# Autodesk Inventor assembly: Robot
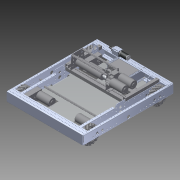
[picture p0: Inventor's stored thumbnail of the model, 180x180]
Saved by Autodesk Inventor 2015 SP1 (Build 190203100, 203)
## iProperties
Created: 2015-01-10
Part Number: Robot
Document SubType Name: Assembly
Designer: Jarod
Author: Jarod
## Documents named in this file (29)
- C:\Users\Jarod\Documents\Westview\Robotics\FRC\2015\CAD\Robot\Chassis\Chassis.iam
- C:\Users\Jarod\Documents\Westview\Robotics\FRC\2015\CAD\Robot\Chassis\Imported Components\AM14U2 End Sheet\AM14U2 End Sheet.ipt
- C:\Users\Jarod\Documents\Westview\Robotics\FRC\2015\CAD\Robot\Chassis\Imported Components\AM14U2 Inside Sheet\AM14U2 Inside Sheet.ipt
- C:\Users\Jarod\Documents\Westview\Robotics\FRC\2015\CAD\Robot\Chassis\Imported Components\AM14U2 Outside Sheet\AM14U2 Outside Sheet.ipt
- C:\Users\Jarod\Documents\Westview\Robotics\FRC\2015\CAD\Robot\Chassis\Imported Components\hub hex 0.5in\hub hex 0.5in.ipt
- C:\Users\Jarod\Documents\Westview\Robotics\FRC\2015\CAD\Robot\Chassis\Imported Components\Toughbox nano hex\Toughbox nano hex.iam
- C:\Users\Jarod\Documents\Westview\Robotics\FRC\2015\CAD\Robot\Chassis\ToughBox Nano Mounting Plate.ipt
- C:\Users\Jarod\Documents\Westview\Robotics\FRC\2015\CAD\Robot\Chassis\Imported Components\mecanum 6in left\mecanum 6in left.iam
- C:\Users\Jarod\Documents\Westview\Robotics\FRC\2015\CAD\Robot\Chassis\Imported Components\mecanum 6in right\mecanum 6in right.iam
- C:\Users\Jarod\Documents\Westview\Robotics\FRC\2015\CAD\Robot\Chassis\Imported Components\Battery Holder\Battery Holder.iam
- C:\Users\Jarod\Documents\Westview\Robotics\FRC\2015\CAD\Robot\Chassis\battery.ipt
- C:\Users\Jarod\Documents\Westview\Robotics\FRC\2015\CAD\Robot\Chassis\polycarb base.ipt
- C:\Users\Jarod\Documents\Westview\Robotics\FRC\2015\CAD\Robot\Chassis\churro.ipt
- C:\Users\Jarod\Documents\Westview\Robotics\FRC\2015\CAD\Robot\Chassis\churro long.ipt
- C:\Users\Jarod\Documents\Westview\Robotics\FRC\2015\CAD\Robot\Chassis\Imported Components\Versaplanetary Gearbox\Versaplanetary Gearbox.iam
- C:\Users\Jarod\Documents\Westview\Robotics\FRC\2015\CAD\Robot\Chassis\Imported Components\0.5 Hex #25 Chain 16t Sprocket\0.5 Hex #25 Chain 16t Sprocket.ipt
- C:\Users\Jarod\Documents\Westview\Robotics\FRC\2015\CAD\Robot\Chassis\Imported Components\0.5 Hex Shaft Collar\0.5 Hex Shaft Collar.ipt
- C:\Users\Jarod\Documents\Westview\Robotics\FRC\2015\CAD\Robot\Chassis\mounting block.ipt
- C:\Users\Jarod\Documents\Westview\Robotics\FRC\2015\CAD\Robot\Chassis\Imported Components\Bearing Side Gusset\Bearing Side Gusset.ipt
- C:\Users\Jarod\Documents\Westview\Robotics\FRC\2015\CAD\Robot\Chassis\mounting block long.ipt
- C:\Users\Jarod\Documents\Westview\Robotics\FRC\2015\CAD\Robot\Chassis\Imported Components\Toughbox-mini\Toughbox-mini.iam
- C:\Users\Jarod\Documents\Westview\Robotics\FRC\2015\CAD\Robot\Chassis\Imported Components\Toughbox-mini\Toughbox-mini_d02.ipt
- C:\Users\Jarod\Documents\Westview\Robotics\FRC\2015\CAD\Robot\Chassis\Imported Components\0.5 Hex Bearing\0.5 Hex Bearing.ipt
- C:\Users\Jarod\Documents\Westview\Robotics\FRC\2015\CAD\Robot\Chassis\Imported Components\0.5 hex coupler\0.5 hex coupler.iam
- C:\Users\Jarod\Documents\Westview\Robotics\FRC\2015\CAD\Robot\Chassis\Imported Components\Toughbox nano hex\CIM motor.ipt
- C:\Users\Jarod\Documents\Westview\Robotics\FRC\2015\CAD\Robot\Chassis\churro gearbox support.ipt
- C:\Users\Jarod\Documents\Westview\Robotics\FRC\2015\CAD\Robot\Chassis\0.5 hex shaft.ipt
- C:\Users\Jarod\Documents\Westview\Robotics\FRC\2015\CAD\Robot\Chassis\2in spool roller.ipt
- C:\Users\Jarod\Documents\Westview\Robotics\FRC\2015\CAD\Robot\Chassis\spool roller hub.ipt
## Components (53 placed, 28 different names)
1. AM14U2 End Sheet:1 — Mate:1, Flush:1, Flush:2, Mate:2, Mate:12, Mate:13, Mate:14, Mate:15, Mate:16, Mate:17, Mate:18, Mate:54, Mate:56, Mate:58, Mate:59, Mate:60, Mate:61, Mate:72, Mate:73
2. AM14U2 End Sheet:2 — Mate:19, Mate:20, Mate:21, Mate:55, Mate:57, Mate:66, Mate:67, Mate:68, Mate:70, Mate:94
3. AM14U2 Inside Sheet:1 — Mate:12, Mate:47, Mate:49, Flush:7, Flush:8, Mate:60, Mate:61, Mate:62, Mate:63, Flush:11, Mate:74, Mate:75, Mate:78, Mate:79, Mate:82, Mate:83, Mate:84, Mate:85, Mate:122, Mate:139, Mate:151, Mate:152, Mate:153, Mate:155, Mate:156
4. AM14U2 Inside Sheet:2 — Mate:2, Mate:46, Mate:48, Flush:9, Flush:10, Mate:58, Mate:59, Mate:64, Mate:65, Mate:76, Mate:77, Mate:80, Mate:81, Mate:125, Mate:140, Mate:154, Mate:157, Mate:158
5. AM14U2 Outside Sheet:1 — Mate:13, Mate:14, Mate:15, Mate:19, Mate:20, Mate:21
6. AM14U2 Outside Sheet:2 — Mate:16, Mate:17, Mate:18
7. churro:1 — Mate:74, Mate:79
8. churro:2 — Mate:75, Mate:78
9. churro:3 — Mate:76, Mate:81
10. churro:4 — Mate:77, Mate:80
11. churro long:1 — Mate:82, Mate:84
12. churro long:2 — Mate:83, Mate:85
13. Toughbox nano hex:1 [sub-assembly] — Mate:23, Mate:25, Mate:38, Flush:3, Mate:39, Mate:54, Flush:7
14. Toughbox nano hex:2 [sub-assembly] — Mate:26, Mate:29, Mate:40, Flush:4, Mate:41, Mate:55, Flush:8
15. Toughbox nano hex:3 [sub-assembly] — Mate:30, Mate:33, Mate:44, Flush:6, Mate:45, Flush:9, Mate:56
16. Toughbox nano hex:4 [sub-assembly] — Mate:36, Mate:42, Flush:5, Mate:43, Mate:57, Flush:10
17. ToughBox Nano Mounting Plate:1 — Mate:38, Flush:3, Mate:39, Mate:47
18. ToughBox Nano Mounting Plate:2 — Mate:40, Flush:4, Mate:41, Mate:49
19. ToughBox Nano Mounting Plate:3 — Mate:44, Flush:6, Mate:45, Mate:46
20. ToughBox Nano Mounting Plate:4 — Mate:42, Flush:5, Mate:43, Mate:48
21. hub hex 0.5in:1 — Mate:23, Mate:24, Mate:63
22. hub hex 0.5in:2 — Mate:26, Mate:28, Mate:62
23. hub hex 0.5in:3 — Mate:30, Mate:32, Mate:64
24. hub hex 0.5in:4 — Mate:34, Mate:35, Mate:36, Mate:65
25. mecanum 6in left:1 [sub-assembly] — Mate:24, Mate:25
26. mecanum 6in left:2 [sub-assembly] — Mate:34, Mate:35
27. mecanum 6in right:1 [sub-assembly] — Mate:28, Mate:29
28. mecanum 6in right:2 [sub-assembly] — Mate:32, Mate:33
29. Battery Holder:1 [sub-assembly] — Mate:66, Mate:67, Mate:68, Mate:69, Mate:71, Mate:114, Mate:115
30. battery:1 — Mate:69, Mate:70, Mate:71
31. polycarb base:1 — Mate:72, Flush:11, Mate:73
32. Versaplanetary Gearbox:1 [sub-assembly] — Mate:94, Mate:97, Mate:100, Mate:114, Mate:115
33. 0.5 Hex #25 Chain 16t Sprocket:1 — Mate:97, Mate:98, Mate:99, Mate:100
34. 0.5 Hex Shaft Collar:1 — Mate:98, Mate:99
35. mounting block:1 — Mate:122, Mate:131, Mate:132, Mate:133, Mate:155, Mate:156
36. mounting block:2 — Mate:125, Mate:128, Mate:129, Mate:130, Mate:157, Mate:158
37. Bearing Side Gusset:1 — Mate:131, Mate:132, Mate:133
38. Bearing Side Gusset:2 — Mate:128, Mate:129, Mate:130
39. mounting block long:1 — Mate:141, Mate:142, Mate:152, Mate:153, Mate:154, Mate:164, Mate:165
40. mounting block long:2 — Mate:139, Mate:140, Mate:151, Mate:163, Mate:166
41. Toughbox-mini:1 [sub-assembly] — Mate:141, Mate:147, Mate:148, Mate:149, Mate:159, Mate:160, Mate:161, Mate:162, Mate:163, Mate:164, Mate:167, Mate:168, Mate:169, Mate:170, Mate:171, Mate:178
42. Toughbox-mini_d02:1 — Mate:142, Mate:145, Mate:146, Mate:165, Mate:166
43. 0.5 Hex Bearing:1 — Mate:145, Mate:146, Mate:174, Mate:175
44. 0.5 hex coupler:1 [sub-assembly] — Mate:147, Mate:148, Mate:149, Mate:172, Mate:173, Mate:179
45. CIM motor:1 — Mate:159, Mate:161
46. CIM motor:2 — Mate:160, Mate:162
47. churro gearbox support:1 — Mate:167, Mate:170
48. churro gearbox support:2 — Mate:168, Mate:169
49. 0.5 hex shaft:1 — Mate:171, Mate:172, Mate:173
50. 0.5 Hex Shaft Collar:2 — Mate:174, Mate:175
51. 2in spool roller:1 — Mate:176, Flush:12, Flush:13, Mate:177, Mate:178
52. spool roller hub:1 — Mate:176, Flush:13, Mate:179
53. spool roller hub:2 — Flush:12, Mate:177
## Relationships (134: Mate 121, Flush 13)
- Mate:1: AM14U2 End Sheet:1
- Flush:1: AM14U2 End Sheet:1
- Flush:2: AM14U2 End Sheet:1
- Mate:2: AM14U2 End Sheet:1 ↔ AM14U2 Inside Sheet:2
- Mate:12: AM14U2 End Sheet:1 ↔ AM14U2 Inside Sheet:1
- Mate:13: AM14U2 End Sheet:1 ↔ AM14U2 Outside Sheet:1
- Mate:14: AM14U2 End Sheet:1 ↔ AM14U2 Outside Sheet:1
- Mate:15: AM14U2 End Sheet:1 ↔ AM14U2 Outside Sheet:1
- Mate:16: AM14U2 End Sheet:1 ↔ AM14U2 Outside Sheet:2
- Mate:17: AM14U2 End Sheet:1 ↔ AM14U2 Outside Sheet:2
- Mate:18: AM14U2 End Sheet:1 ↔ AM14U2 Outside Sheet:2
- Mate:19: AM14U2 End Sheet:2 ↔ AM14U2 Outside Sheet:1
- Mate:20: AM14U2 End Sheet:2 ↔ AM14U2 Outside Sheet:1
- Mate:21: AM14U2 End Sheet:2 ↔ AM14U2 Outside Sheet:1
- Mate:23: Toughbox nano hex:1 ↔ hub hex 0.5in:1
- Mate:24: hub hex 0.5in:1 ↔ mecanum 6in left:1
- Mate:25: Toughbox nano hex:1 ↔ mecanum 6in left:1
- Mate:26: Toughbox nano hex:2 ↔ hub hex 0.5in:2
- Mate:28: hub hex 0.5in:2 ↔ mecanum 6in right:1
- Mate:29: Toughbox nano hex:2 ↔ mecanum 6in right:1
- Mate:30: Toughbox nano hex:3 ↔ hub hex 0.5in:3
- Mate:32: hub hex 0.5in:3 ↔ mecanum 6in right:2
- Mate:33: Toughbox nano hex:3 ↔ mecanum 6in right:2
- Mate:34: hub hex 0.5in:4 ↔ mecanum 6in left:2
- Mate:35: hub hex 0.5in:4 ↔ mecanum 6in left:2
- Mate:36: Toughbox nano hex:4 ↔ hub hex 0.5in:4
- Mate:38: Toughbox nano hex:1 ↔ ToughBox Nano Mounting Plate:1
- Flush:3: Toughbox nano hex:1 ↔ ToughBox Nano Mounting Plate:1
- Mate:39: Toughbox nano hex:1 ↔ ToughBox Nano Mounting Plate:1
- Mate:40: Toughbox nano hex:2 ↔ ToughBox Nano Mounting Plate:2
- Flush:4: Toughbox nano hex:2 ↔ ToughBox Nano Mounting Plate:2
- Mate:41: Toughbox nano hex:2 ↔ ToughBox Nano Mounting Plate:2
- Mate:42: Toughbox nano hex:4 ↔ ToughBox Nano Mounting Plate:4
- Flush:5: Toughbox nano hex:4 ↔ ToughBox Nano Mounting Plate:4
- Mate:43: Toughbox nano hex:4 ↔ ToughBox Nano Mounting Plate:4
- Mate:44: Toughbox nano hex:3 ↔ ToughBox Nano Mounting Plate:3
- Flush:6: Toughbox nano hex:3 ↔ ToughBox Nano Mounting Plate:3
- Mate:45: Toughbox nano hex:3 ↔ ToughBox Nano Mounting Plate:3
- Mate:46: AM14U2 Inside Sheet:2 ↔ ToughBox Nano Mounting Plate:3
- Mate:47: AM14U2 Inside Sheet:1 ↔ ToughBox Nano Mounting Plate:1
- Mate:48: AM14U2 Inside Sheet:2 ↔ ToughBox Nano Mounting Plate:4
- Mate:49: AM14U2 Inside Sheet:1 ↔ ToughBox Nano Mounting Plate:2
- Mate:54 (64.6176 mm): AM14U2 End Sheet:1 ↔ Toughbox nano hex:1
- Flush:7 (-24.4856 mm): AM14U2 Inside Sheet:1 ↔ Toughbox nano hex:1
- Mate:55 (64.6176 mm): AM14U2 End Sheet:2 ↔ Toughbox nano hex:2
- Flush:8 (-24.4856 mm): AM14U2 Inside Sheet:1 ↔ Toughbox nano hex:2
- Flush:9 (-24.4856 mm): AM14U2 Inside Sheet:2 ↔ Toughbox nano hex:3
- Mate:56 (64.6176 mm): AM14U2 End Sheet:1 ↔ Toughbox nano hex:3
- Mate:57 (64.6176 mm): AM14U2 End Sheet:2 ↔ Toughbox nano hex:4
- Flush:10 (-24.4856 mm): AM14U2 Inside Sheet:2 ↔ Toughbox nano hex:4
- Mate:58: AM14U2 End Sheet:1 ↔ AM14U2 Inside Sheet:2
- Mate:59: AM14U2 End Sheet:1 ↔ AM14U2 Inside Sheet:2
- Mate:60: AM14U2 End Sheet:1 ↔ AM14U2 Inside Sheet:1
- Mate:61: AM14U2 End Sheet:1 ↔ AM14U2 Inside Sheet:1
- Mate:62: AM14U2 Inside Sheet:1 ↔ hub hex 0.5in:2
- Mate:63: AM14U2 Inside Sheet:1 ↔ hub hex 0.5in:1
- Mate:64: AM14U2 Inside Sheet:2 ↔ hub hex 0.5in:3
- Mate:65: AM14U2 Inside Sheet:2 ↔ hub hex 0.5in:4
- Mate:66: AM14U2 End Sheet:2 ↔ Battery Holder:1
- Mate:67: AM14U2 End Sheet:2 ↔ Battery Holder:1
- Mate:68: AM14U2 End Sheet:2 ↔ Battery Holder:1
- Mate:69: Battery Holder:1 ↔ battery:1
- Mate:70: AM14U2 End Sheet:2 ↔ battery:1
- Mate:71: Battery Holder:1 ↔ battery:1
- Mate:72: AM14U2 End Sheet:1 ↔ polycarb base:1
- Flush:11: AM14U2 Inside Sheet:1 ↔ polycarb base:1
- Mate:73: AM14U2 End Sheet:1 ↔ polycarb base:1
- Mate:74: AM14U2 Inside Sheet:1 ↔ churro:1
- Mate:75: AM14U2 Inside Sheet:1 ↔ churro:2
- Mate:76: AM14U2 Inside Sheet:2 ↔ churro:3
- Mate:77: AM14U2 Inside Sheet:2 ↔ churro:4
- Mate:78: AM14U2 Inside Sheet:1 ↔ churro:2
- Mate:79: AM14U2 Inside Sheet:1 ↔ churro:1
- Mate:80: AM14U2 Inside Sheet:2 ↔ churro:4
- Mate:81: AM14U2 Inside Sheet:2 ↔ churro:3
- Mate:82: AM14U2 Inside Sheet:1 ↔ churro long:1
- Mate:83: AM14U2 Inside Sheet:1 ↔ churro long:2
- Mate:84: AM14U2 Inside Sheet:1 ↔ churro long:1
- Mate:85: AM14U2 Inside Sheet:1 ↔ churro long:2
- Mate:94: AM14U2 End Sheet:2 ↔ Versaplanetary Gearbox:1
- Mate:97: Versaplanetary Gearbox:1 ↔ 0.5 Hex #25 Chain 16t Sprocket:1
- Mate:98: 0.5 Hex #25 Chain 16t Sprocket:1 ↔ 0.5 Hex Shaft Collar:1
- Mate:99: 0.5 Hex #25 Chain 16t Sprocket:1 ↔ 0.5 Hex Shaft Collar:1
- Mate:100: Versaplanetary Gearbox:1 ↔ 0.5 Hex #25 Chain 16t Sprocket:1
- Mate:114: Battery Holder:1 ↔ Versaplanetary Gearbox:1
- Mate:115: Battery Holder:1 ↔ Versaplanetary Gearbox:1
- Mate:122: AM14U2 Inside Sheet:1 ↔ mounting block:1
- Mate:125: AM14U2 Inside Sheet:2 ↔ mounting block:2
- Mate:128: mounting block:2 ↔ Bearing Side Gusset:2
- Mate:129: mounting block:2 ↔ Bearing Side Gusset:2
- Mate:130: mounting block:2 ↔ Bearing Side Gusset:2
- Mate:131: mounting block:1 ↔ Bearing Side Gusset:1
- Mate:132: mounting block:1 ↔ Bearing Side Gusset:1
- Mate:133: mounting block:1 ↔ Bearing Side Gusset:1
- Mate:139: AM14U2 Inside Sheet:1 ↔ mounting block long:2
- Mate:140: AM14U2 Inside Sheet:2 ↔ mounting block long:2
- Mate:141: mounting block long:1 ↔ Toughbox-mini:1
- Mate:142: mounting block long:1 ↔ Toughbox-mini_d02:1
- Mate:145: Toughbox-mini_d02:1 ↔ 0.5 Hex Bearing:1
- Mate:146: Toughbox-mini_d02:1 ↔ 0.5 Hex Bearing:1
- Mate:147: Toughbox-mini:1 ↔ 0.5 hex coupler:1
- Mate:148: Toughbox-mini:1 ↔ 0.5 hex coupler:1
- Mate:149 (-19.05 mm): Toughbox-mini:1 ↔ 0.5 hex coupler:1
- Mate:151: AM14U2 Inside Sheet:1 ↔ mounting block long:2
- Mate:152: AM14U2 Inside Sheet:1 ↔ mounting block long:1
- Mate:153: AM14U2 Inside Sheet:1 ↔ mounting block long:1
- Mate:154: AM14U2 Inside Sheet:2 ↔ mounting block long:1
- Mate:155: AM14U2 Inside Sheet:1 ↔ mounting block:1
- Mate:156: AM14U2 Inside Sheet:1 ↔ mounting block:1
- Mate:157: AM14U2 Inside Sheet:2 ↔ mounting block:2
- Mate:158: AM14U2 Inside Sheet:2 ↔ mounting block:2
- Mate:159: Toughbox-mini:1 ↔ CIM motor:1
- Mate:160: Toughbox-mini:1 ↔ CIM motor:2
- Mate:161: Toughbox-mini:1 ↔ CIM motor:1
- Mate:162: Toughbox-mini:1 ↔ CIM motor:2
- Mate:163: mounting block long:2 ↔ Toughbox-mini:1
- Mate:164: mounting block long:1 ↔ Toughbox-mini:1
- Mate:165: mounting block long:1 ↔ Toughbox-mini_d02:1
- Mate:166: mounting block long:2 ↔ Toughbox-mini_d02:1
- Mate:167: Toughbox-mini:1 ↔ churro gearbox support:1
- Mate:168: Toughbox-mini:1 ↔ churro gearbox support:2
- Mate:169: Toughbox-mini:1 ↔ churro gearbox support:2
- Mate:170: Toughbox-mini:1 ↔ churro gearbox support:1
- Mate:171: Toughbox-mini:1 ↔ 0.5 hex shaft:1
- Mate:172: 0.5 hex coupler:1 ↔ 0.5 hex shaft:1
- Mate:173: 0.5 hex coupler:1 ↔ 0.5 hex shaft:1
- Mate:174: 0.5 Hex Bearing:1 ↔ 0.5 Hex Shaft Collar:2
- Mate:175: 0.5 Hex Bearing:1 ↔ 0.5 Hex Shaft Collar:2
- Mate:176: 2in spool roller:1 ↔ spool roller hub:1
- Flush:12: 2in spool roller:1 ↔ spool roller hub:2
- Flush:13: 2in spool roller:1 ↔ spool roller hub:1
- Mate:177: 2in spool roller:1 ↔ spool roller hub:2
- Mate:178: Toughbox-mini:1 ↔ 2in spool roller:1
- Mate:179: 0.5 hex coupler:1 ↔ spool roller hub:1
